# Autodesk Inventor assembly: IMUTracker_assemble
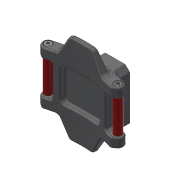
[picture p0: Inventor's stored thumbnail of the model, 180x180]
Saved by Autodesk Inventor 2019.4 (Build 234330000, 330)
## iProperties
Created: 2019-11-17
Part Number: IMUTracker_assemble
Material: 一般
Document SubType Name: Assembly
Designer: y6tada
Author: y6tada
## Documents named in this file (7)
- C:\Workspace\QUIKS\Hardware\IMUTracker\Casing\Single\IMUTracker_assemble.iam
- C:\Workspace\QUIKS\Hardware\IMUTracker\Casing\Single\IMUTracker_casing_v2.ipt
- C:\Workspace\QUIKS\Hardware\IMUTracker\Casing\Single\AR-2622.ipt
- C:\Users\y6tada\Documents\Inventor\Content Center Files\R2019\ja-JP\ISO 4762(2)\ISO 4762 - M2.5 x 10ISO.ipt
- C:\Workspace\QUIKS\Hardware\IMUTracker\Circuit\IMUTracker.iam
- C:\Workspace\QUIKS\Hardware\QUIKS_SINGLE_COVER.ipt
- C:\Workspace\QUIKS\Hardware\IMUTracker\Casing\Single\C-2003-4.ipt
## Components (13 placed, 6 different names)
1. IMUTracker_casing_v2:1 — メイト:4, メイト:5, メイト:6, メイト:7, 挿入:1, 挿入:2, 挿入:3, 挿入:4, メイト:9, メイト:12, メイト:13, メイト:14, メイト:16
2. AR-2622:1 — メイト:4, メイト:5
3. AR-2622:2 — メイト:6, メイト:7
4. ISO 4762 M2.5 x 10:1 — 挿入:1
5. ISO 4762 M2.5 x 10:2 — 挿入:2
6. ISO 4762 M2.5 x 10:3 — 挿入:3
7. ISO 4762 M2.5 x 10:4 — 挿入:4
8. IMUTracker:1 [sub-assembly] — フラッシュ:1, メイト:8, メイト:9, メイト:15, メイト:17, メイト:18, メイト:19
9. QUIKS_SINGLE_COVER:1 — メイト:10, フラッシュ:4, メイト:20
10. C-2003-4:1 — メイト:13, メイト:18, メイト:20
11. C-2003-4:2 — メイト:14, メイト:19
12. C-2003-4:3 — メイト:15, メイト:16
13. C-2003-4:4 — メイト:12, メイト:17
## Relationships (22: Mate 16, Insert 4, Flush 2)
- メイト:4 [Mate]: IMUTracker_casing_v2:1 ↔ AR-2622:1
- メイト:5 [Mate]: IMUTracker_casing_v2:1 ↔ AR-2622:1
- メイト:6 [Mate]: IMUTracker_casing_v2:1 ↔ AR-2622:2
- メイト:7 [Mate]: IMUTracker_casing_v2:1 ↔ AR-2622:2
- 挿入:1 [Insert]: IMUTracker_casing_v2:1 ↔ ISO 4762 M2.5 x 10:1
- 挿入:2 [Insert]: IMUTracker_casing_v2:1 ↔ ISO 4762 M2.5 x 10:2
- 挿入:3 [Insert]: IMUTracker_casing_v2:1 ↔ ISO 4762 M2.5 x 10:3
- 挿入:4 [Insert]: IMUTracker_casing_v2:1 ↔ ISO 4762 M2.5 x 10:4
- フラッシュ:1 [Flush]: IMUTracker:1
- メイト:8 [Mate]: IMUTracker:1
- メイト:9 [Mate]: IMUTracker_casing_v2:1 ↔ IMUTracker:1
- メイト:10 [Mate]: QUIKS_SINGLE_COVER:1
- フラッシュ:4 [Flush]: QUIKS_SINGLE_COVER:1
- メイト:12 [Mate]: IMUTracker_casing_v2:1 ↔ C-2003-4:4
- メイト:13 [Mate]: IMUTracker_casing_v2:1 ↔ C-2003-4:1
- メイト:14 [Mate]: IMUTracker_casing_v2:1 ↔ C-2003-4:2
- メイト:15 [Mate]: IMUTracker:1 ↔ C-2003-4:3
- メイト:16 [Mate]: IMUTracker_casing_v2:1 ↔ C-2003-4:3
- メイト:17 [Mate]: IMUTracker:1 ↔ C-2003-4:4
- メイト:18 [Mate]: IMUTracker:1 ↔ C-2003-4:1
- メイト:19 [Mate]: IMUTracker:1 ↔ C-2003-4:2
- メイト:20 [Mate]: QUIKS_SINGLE_COVER:1 ↔ C-2003-4:1
